# Autodesk Inventor assembly: Indexer 2.0 MASTER
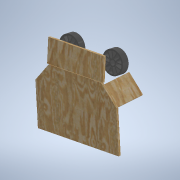
[picture p0: Inventor's stored thumbnail of the model, 180x180]
Saved by Autodesk Inventor 2020 (Build 240168000, 168)
## iProperties
Created: 2020-01-25
Part Number: Indexer 2.0 MASTER
Document SubType Name: Assembly
Designer: 1cikaychapman
Author: 1cikaychapman
## Documents named in this file (5)
- C:\Users\autum\Google Drive\Iron Riders 4180 (Roosevelt Robotics)\2019-2020\Build_Design\Robot 2020 (1)\Indexer 2.0\Indexer 2.0 MASTER.iam
- C:\Users\autum\Google Drive\Iron Riders 4180 (Roosevelt Robotics)\2019-2020\Build_Design\Robot 2020 (1)\Indexer 2.0\Slope.ipt
- C:\Users\autum\Google Drive\Iron Riders 4180 (Roosevelt Robotics)\2019-2020\Build_Design\Robot 2020 (1)\Indexer 2.0\Flat Section.ipt
- C:\Users\autum\Google Drive\Iron Riders 4180 (Roosevelt Robotics)\2019-2020\Build_Design\Robot 2020 (1)\Indexer 2.0\5_Straight_Flex_Wheel_60A_217-6455.ipt
- C:\Users\autum\Google Drive\Iron Riders 4180 (Roosevelt Robotics)\2019-2020\Build_Design\Robot 2020 (1)\Indexer 2.0\Side slant.ipt
## Components (6 placed, 4 different names)
1. Slope:1 — Flush:1, Angle:1, Mate:13, Mate:15, Flush:6, Flush:7, Mate:16, Mate:17, Mate:18
2. Flat Section:1 — Flush:1, Mate:2, Mate:3, Mate:5, Mate:6, Mate:7, Angle:1, Mate:16
3. 5_Straight_Flex_Wheel_60A_217-6455:1 — Mate:2, Mate:4, Mate:5, Mate:6
4. 5_Straight_Flex_Wheel_60A_217-6455:2 — Mate:3, Mate:4, Mate:7
5. Side slant:1 — Mate:15, Flush:6, Mate:18
6. Side slant:2 — Mate:13, Flush:7, Mate:17
## Relationships (15: Mate 11, Flush 3, Angle 1)
- Flush:1 (76.2 mm): Slope:1 ↔ Flat Section:1
- Mate:2 (88.9 mm): Flat Section:1 ↔ 5_Straight_Flex_Wheel_60A_217-6455:1
- Mate:3 (88.9 mm): Flat Section:1 ↔ 5_Straight_Flex_Wheel_60A_217-6455:2
- Mate:4 (266.7 mm): 5_Straight_Flex_Wheel_60A_217-6455:1 ↔ 5_Straight_Flex_Wheel_60A_217-6455:2
- Mate:5 (-38.1 mm): Flat Section:1 ↔ 5_Straight_Flex_Wheel_60A_217-6455:1
- Mate:6 (-63.5 mm): Flat Section:1 ↔ 5_Straight_Flex_Wheel_60A_217-6455:1
- Mate:7 (-63.5 mm): Flat Section:1 ↔ 5_Straight_Flex_Wheel_60A_217-6455:2
- Angle:1 (7.5 deg): Slope:1 ↔ Flat Section:1
- Mate:13: Slope:1 ↔ Side slant:2
- Mate:15: Slope:1 ↔ Side slant:1
- Flush:6: Slope:1 ↔ Side slant:1
- Flush:7: Slope:1 ↔ Side slant:2
- Mate:16: Slope:1 ↔ Flat Section:1
- Mate:17: Slope:1 ↔ Side slant:2
- Mate:18: Slope:1 ↔ Side slant:1
